# Autodesk Inventor assembly: 42146-19
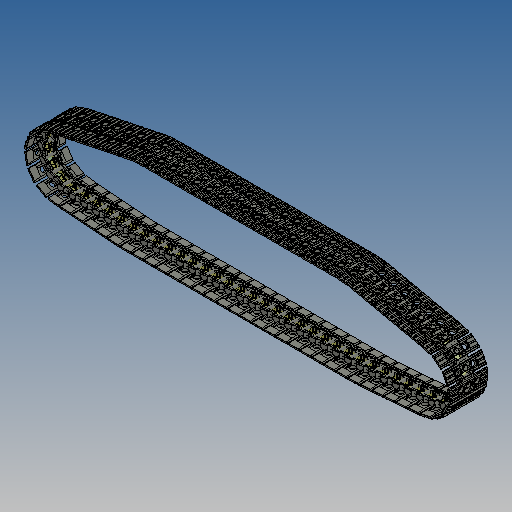
[picture p0: Inventor's stored thumbnail of the model, 512x512]
Saved by Autodesk Inventor 2025 (Build 290162010, 162A)
## iProperties
Created: 2024-11-19
Part Number: 42146-19
Material: Generisch
Document SubType Name: Assembly
Designer: hp.muther
Author: hp.muther
## Documents named in this file (3)
- D:\Inventor\Projekte\Muther\LEGO Technic\LEGO Technik - Raupenkran LR 13000 (42146)\42146-19.iam
- D:\Inventor\Projekte\Muther\LEGO Technic\LEGO Technik - Raupenkran LR 13000 (42146)\42146-19.ipt
- D:\Inventor\Projekte\Muther\LEGO Technic\LEGO Pieces\Räder, Raupe\57518-DkBluishGray.ipt
## Components (76 placed, 2 different names)
1. 42146-19:1 — Passend:1, Passend:2, Passend:3, Passend:4, Passend:5, Passend:6, Passend:7, Tangential:1, Tangential:2, Tangential:3, Tangential:4, Tangential:5, Tangential:6, Passend:8, Passend:9, Passend:10, Passend:11, Passend:12, Passend:13, Passend:14, Passend:15, Passend:16, Passend:17, Passend:18, Passend:19, Passend:20, Passend:21, Passend:22, Passend:23, Passend:24, Passend:25, Passend:26, Passend:27, Passend:28, Passend:29, Passend:30, Passend:31, Passend:32, Passend:33, Passend:34, Passend:35, Passend:36, Passend:37, Passend:38, Passend:39, Passend:40, Tangential:7, Tangential:8, Tangential:9, Tangential:10, Tangential:11, Tangential:12, Passend:41, Passend:42, Passend:43, Passend:44, Passend:45, Passend:46, Passend:47, Passend:48, Passend:49, Passend:50, Passend:51, Passend:52, Passend:53, Passend:54, Passend:55, Passend:56, Passend:57, Passend:58, Passend:59, Passend:60, Passend:61, Passend:62, Passend:63, Passend:64, Passend:65
2. 57518-DkBluishGray:1 — Passend:1, Passend:2, Passend:3, Einfügen:1
3. 57518-DkBluishGray:2 — Einfügen:1, Einfügen:3, Passend:4
4. 57518-DkBluishGray:3 — Einfügen:3, Passend:5
5. 57518-DkBluishGray:4 — Einfügen:7, Passend:6
6. 57518-DkBluishGray:5 — Einfügen:7, Passend:7
7. 57518-DkBluishGray:6 — Passend:10
8. 57518-DkBluishGray:7 — Tangential:1
9. 57518-DkBluishGray:8 — Einfügen:15, Tangential:2
10. 57518-DkBluishGray:9 — Einfügen:15, Tangential:3
11. 57518-DkBluishGray:10 — Tangential:4
12. 57518-DkBluishGray:11 — Tangential:5
13. 57518-DkBluishGray:12 — Tangential:6
14. 57518-DkBluishGray:13 — Passend:8
15. 57518-DkBluishGray:14 — Passend:9
16. 57518-DkBluishGray:15 — Passend:11
17. 57518-DkBluishGray:16 — Passend:12, Einfügen:31
18. 57518-DkBluishGray:17 — Einfügen:31, Passend:13
19. 57518-DkBluishGray:18 — Passend:14
20. 57518-DkBluishGray:19 — Passend:15
21. 57518-DkBluishGray:20 — Passend:16
22. 57518-DkBluishGray:21 — Passend:17
23. 57518-DkBluishGray:22 — Passend:18
24. 57518-DkBluishGray:23 — Passend:19
25. 57518-DkBluishGray:24 — Passend:20
26. 57518-DkBluishGray:25 — Passend:21
27. 57518-DkBluishGray:26 — Passend:22
28. 57518-DkBluishGray:27 — Passend:23
29. 57518-DkBluishGray:28 — Passend:24
30. 57518-DkBluishGray:29 — Passend:25
31. 57518-DkBluishGray:30 — Passend:26
32. 57518-DkBluishGray:31 — Passend:27
33. 57518-DkBluishGray:32 — Passend:28, Einfügen:63
34. 57518-DkBluishGray:33 — Einfügen:63, Passend:29
35. 57518-DkBluishGray:34 — Passend:30
36. 57518-DkBluishGray:35 — Passend:31
37. 57518-DkBluishGray:36 — Passend:32
38. 57518-DkBluishGray:37 — Passend:33
39. 57518-DkBluishGray:38 — Passend:34
40. 57518-DkBluishGray:39 — Passend:35
41. 57518-DkBluishGray:40 — Passend:36
42. 57518-DkBluishGray:41 — Passend:37
43. 57518-DkBluishGray:42 — Passend:38
44. 57518-DkBluishGray:43 — Passend:39
45. 57518-DkBluishGray:44 — Passend:40
46. 57518-DkBluishGray:45 — Tangential:7
47. 57518-DkBluishGray:46 — Tangential:8
48. 57518-DkBluishGray:47 — Tangential:9
49. 57518-DkBluishGray:48 — Tangential:10
50. 57518-DkBluishGray:49 — Tangential:11
51. 57518-DkBluishGray:50 — Tangential:12
52. 57518-DkBluishGray:51 — Passend:41
53. 57518-DkBluishGray:52 — Passend:42
54. 57518-DkBluishGray:53 — Passend:43
55. 57518-DkBluishGray:54 — Passend:44
56. 57518-DkBluishGray:55 — Passend:45
57. 57518-DkBluishGray:56 — Passend:46
58. 57518-DkBluishGray:57 — Passend:47
59. 57518-DkBluishGray:58 — Passend:48
60. 57518-DkBluishGray:59 — Passend:49
61. 57518-DkBluishGray:60 — Passend:50
62. 57518-DkBluishGray:61 — Passend:51
63. 57518-DkBluishGray:62 — Passend:52
64. 57518-DkBluishGray:63 — Passend:53
65. 57518-DkBluishGray:64 — Passend:54, Einfügen:75
66. 57518-DkBluishGray:65 — Einfügen:75, Passend:55
67. 57518-DkBluishGray:66 — Passend:56
68. 57518-DkBluishGray:67 — Passend:57
69. 57518-DkBluishGray:68 — Passend:58
70. 57518-DkBluishGray:69 — Passend:59
71. 57518-DkBluishGray:70 — Passend:61
72. 57518-DkBluishGray:71 — Passend:60
73. 57518-DkBluishGray:72 — Passend:62
74. 57518-DkBluishGray:73 — Passend:63
75. 57518-DkBluishGray:74 — Passend:64
76. 57518-DkBluishGray:75 — Passend:65
## Relationships (151: Insert 74, Mate 65, Tangent 12)
- Passend:1 [Mate] (-19.2 mm): 42146-19:1 ↔ 57518-DkBluishGray:1
- Passend:2 [Mate]: 42146-19:1 ↔ 57518-DkBluishGray:1
- Passend:3 [Mate]: 42146-19:1 ↔ 57518-DkBluishGray:1
- Einfügen:1 [Insert]: 57518-DkBluishGray:1 ↔ 57518-DkBluishGray:2
- [Insert]: 57518-DkBluishGray:3 ↔ 57518-DkBluishGray:4
- Einfügen:3 [Insert]: 57518-DkBluishGray:2 ↔ 57518-DkBluishGray:3
- [Insert]: 57518-DkBluishGray:5 ↔ 57518-DkBluishGray:6
- [Insert]: 57518-DkBluishGray:7 ↔ 57518-DkBluishGray:8
- [Insert]: 57518-DkBluishGray:6 ↔ 57518-DkBluishGray:7
- Einfügen:7 [Insert]: 57518-DkBluishGray:4 ↔ 57518-DkBluishGray:5
- [Insert]: 57518-DkBluishGray:9 ↔ 57518-DkBluishGray:10
- [Insert]: 57518-DkBluishGray:11 ↔ 57518-DkBluishGray:12
- [Insert]: 57518-DkBluishGray:10 ↔ 57518-DkBluishGray:11
- [Insert]: 57518-DkBluishGray:13 ↔ 57518-DkBluishGray:14
- [Insert]: 57518-DkBluishGray:15 ↔ 57518-DkBluishGray:16
- [Insert]: 57518-DkBluishGray:14 ↔ 57518-DkBluishGray:15
- [Insert]: 57518-DkBluishGray:12 ↔ 57518-DkBluishGray:13
- Einfügen:15 [Insert]: 57518-DkBluishGray:8 ↔ 57518-DkBluishGray:9
- Passend:4 [Mate]: 42146-19:1 ↔ 57518-DkBluishGray:2
- Passend:5 [Mate]: 42146-19:1 ↔ 57518-DkBluishGray:3
- Passend:6 [Mate]: 42146-19:1 ↔ 57518-DkBluishGray:4
- Passend:7 [Mate]: 42146-19:1 ↔ 57518-DkBluishGray:5
- Tangential:1 (-1.6 mm): 42146-19:1 ↔ 57518-DkBluishGray:7
- Tangential:2 (-1.6 mm): 42146-19:1 ↔ 57518-DkBluishGray:8
- Tangential:3 (-1.6 mm): 42146-19:1 ↔ 57518-DkBluishGray:9
- Tangential:4 (-1.6 mm): 42146-19:1 ↔ 57518-DkBluishGray:10
- Tangential:5 (-1.6 mm): 42146-19:1 ↔ 57518-DkBluishGray:11
- Tangential:6 (-1.6 mm): 42146-19:1 ↔ 57518-DkBluishGray:12
- Passend:8 [Mate]: 42146-19:1 ↔ 57518-DkBluishGray:13
- Passend:9 [Mate]: 42146-19:1 ↔ 57518-DkBluishGray:14
- Passend:10 [Mate]: 42146-19:1 ↔ 57518-DkBluishGray:6
- Passend:11 [Mate]: 42146-19:1 ↔ 57518-DkBluishGray:15
- Passend:12 [Mate]: 42146-19:1 ↔ 57518-DkBluishGray:16
- [Insert]: 57518-DkBluishGray:17 ↔ 57518-DkBluishGray:18
- [Insert]: 57518-DkBluishGray:19 ↔ 57518-DkBluishGray:20
- [Insert]: 57518-DkBluishGray:18 ↔ 57518-DkBluishGray:19
- [Insert]: 57518-DkBluishGray:21 ↔ 57518-DkBluishGray:22
- [Insert]: 57518-DkBluishGray:23 ↔ 57518-DkBluishGray:24
- [Insert]: 57518-DkBluishGray:22 ↔ 57518-DkBluishGray:23
- [Insert]: 57518-DkBluishGray:20 ↔ 57518-DkBluishGray:21
- [Insert]: 57518-DkBluishGray:25 ↔ 57518-DkBluishGray:26
- [Insert]: 57518-DkBluishGray:27 ↔ 57518-DkBluishGray:28
- [Insert]: 57518-DkBluishGray:26 ↔ 57518-DkBluishGray:27
- [Insert]: 57518-DkBluishGray:29 ↔ 57518-DkBluishGray:30
- [Insert]: 57518-DkBluishGray:31 ↔ 57518-DkBluishGray:32
- [Insert]: 57518-DkBluishGray:30 ↔ 57518-DkBluishGray:31
- [Insert]: 57518-DkBluishGray:28 ↔ 57518-DkBluishGray:29
- [Insert]: 57518-DkBluishGray:24 ↔ 57518-DkBluishGray:25
- Einfügen:31 [Insert]: 57518-DkBluishGray:16 ↔ 57518-DkBluishGray:17
- Passend:13 [Mate]: 42146-19:1 ↔ 57518-DkBluishGray:17
- Passend:14 [Mate]: 42146-19:1 ↔ 57518-DkBluishGray:18
- Passend:15 [Mate]: 42146-19:1 ↔ 57518-DkBluishGray:19
- Passend:16 [Mate]: 42146-19:1 ↔ 57518-DkBluishGray:20
- Passend:17 [Mate]: 42146-19:1 ↔ 57518-DkBluishGray:21
- Passend:18 [Mate]: 42146-19:1 ↔ 57518-DkBluishGray:22
- Passend:19 [Mate]: 42146-19:1 ↔ 57518-DkBluishGray:23
- Passend:20 [Mate]: 42146-19:1 ↔ 57518-DkBluishGray:24
- Passend:21 [Mate]: 42146-19:1 ↔ 57518-DkBluishGray:25
- Passend:22 [Mate]: 42146-19:1 ↔ 57518-DkBluishGray:26
- Passend:23 [Mate]: 42146-19:1 ↔ 57518-DkBluishGray:27
- Passend:24 [Mate]: 42146-19:1 ↔ 57518-DkBluishGray:28
- Passend:25 [Mate]: 42146-19:1 ↔ 57518-DkBluishGray:29
- Passend:26 [Mate]: 42146-19:1 ↔ 57518-DkBluishGray:30
- Passend:27 [Mate]: 42146-19:1 ↔ 57518-DkBluishGray:31
- Passend:28 [Mate]: 42146-19:1 ↔ 57518-DkBluishGray:32
- [Insert]: 57518-DkBluishGray:33 ↔ 57518-DkBluishGray:34
- [Insert]: 57518-DkBluishGray:35 ↔ 57518-DkBluishGray:36
- [Insert]: 57518-DkBluishGray:34 ↔ 57518-DkBluishGray:35
- [Insert]: 57518-DkBluishGray:37 ↔ 57518-DkBluishGray:38
- [Insert]: 57518-DkBluishGray:39 ↔ 57518-DkBluishGray:40
- [Insert]: 57518-DkBluishGray:38 ↔ 57518-DkBluishGray:39
- [Insert]: 57518-DkBluishGray:36 ↔ 57518-DkBluishGray:37
- [Insert]: 57518-DkBluishGray:41 ↔ 57518-DkBluishGray:42
- [Insert]: 57518-DkBluishGray:43 ↔ 57518-DkBluishGray:44
- [Insert]: 57518-DkBluishGray:42 ↔ 57518-DkBluishGray:43
- [Insert]: 57518-DkBluishGray:45 ↔ 57518-DkBluishGray:46
- [Insert]: 57518-DkBluishGray:47 ↔ 57518-DkBluishGray:48
- [Insert]: 57518-DkBluishGray:46 ↔ 57518-DkBluishGray:47
- [Insert]: 57518-DkBluishGray:44 ↔ 57518-DkBluishGray:45
- [Insert]: 57518-DkBluishGray:40 ↔ 57518-DkBluishGray:41
- [Insert]: 57518-DkBluishGray:49 ↔ 57518-DkBluishGray:50
- [Insert]: 57518-DkBluishGray:51 ↔ 57518-DkBluishGray:52
- [Insert]: 57518-DkBluishGray:50 ↔ 57518-DkBluishGray:51
- [Insert]: 57518-DkBluishGray:53 ↔ 57518-DkBluishGray:54
- [Insert]: 57518-DkBluishGray:55 ↔ 57518-DkBluishGray:56
- [Insert]: 57518-DkBluishGray:54 ↔ 57518-DkBluishGray:55
- [Insert]: 57518-DkBluishGray:52 ↔ 57518-DkBluishGray:53
- [Insert]: 57518-DkBluishGray:57 ↔ 57518-DkBluishGray:58
- [Insert]: 57518-DkBluishGray:59 ↔ 57518-DkBluishGray:60
- [Insert]: 57518-DkBluishGray:58 ↔ 57518-DkBluishGray:59
- [Insert]: 57518-DkBluishGray:61 ↔ 57518-DkBluishGray:62
- [Insert]: 57518-DkBluishGray:63 ↔ 57518-DkBluishGray:64
- [Insert]: 57518-DkBluishGray:62 ↔ 57518-DkBluishGray:63
- [Insert]: 57518-DkBluishGray:60 ↔ 57518-DkBluishGray:61
- [Insert]: 57518-DkBluishGray:56 ↔ 57518-DkBluishGray:57
- [Insert]: 57518-DkBluishGray:48 ↔ 57518-DkBluishGray:49
- Einfügen:63 [Insert]: 57518-DkBluishGray:32 ↔ 57518-DkBluishGray:33
- Passend:29 [Mate]: 42146-19:1 ↔ 57518-DkBluishGray:33
- Passend:30 [Mate]: 42146-19:1 ↔ 57518-DkBluishGray:34
- Passend:31 [Mate]: 42146-19:1 ↔ 57518-DkBluishGray:35
- Passend:32 [Mate]: 42146-19:1 ↔ 57518-DkBluishGray:36
- Passend:33 [Mate]: 42146-19:1 ↔ 57518-DkBluishGray:37
- Passend:34 [Mate]: 42146-19:1 ↔ 57518-DkBluishGray:38
- Passend:35 [Mate]: 42146-19:1 ↔ 57518-DkBluishGray:39
- Passend:36 [Mate]: 42146-19:1 ↔ 57518-DkBluishGray:40
- Passend:37 [Mate]: 42146-19:1 ↔ 57518-DkBluishGray:41
- Passend:38 [Mate]: 42146-19:1 ↔ 57518-DkBluishGray:42
- Passend:39 [Mate]: 42146-19:1 ↔ 57518-DkBluishGray:43
- Passend:40 [Mate]: 42146-19:1 ↔ 57518-DkBluishGray:44
- Tangential:7 (-1.6 mm): 42146-19:1 ↔ 57518-DkBluishGray:45
- Tangential:8 (-1.6 mm): 42146-19:1 ↔ 57518-DkBluishGray:46
- Tangential:9 (-1.6 mm): 42146-19:1 ↔ 57518-DkBluishGray:47
- Tangential:10 (-1.6 mm): 42146-19:1 ↔ 57518-DkBluishGray:48
- Tangential:11 (-1.6 mm): 42146-19:1 ↔ 57518-DkBluishGray:49
- Tangential:12 (-1.6 mm): 42146-19:1 ↔ 57518-DkBluishGray:50
- Passend:41 [Mate]: 42146-19:1 ↔ 57518-DkBluishGray:51
- Passend:42 [Mate]: 42146-19:1 ↔ 57518-DkBluishGray:52
- Passend:43 [Mate]: 42146-19:1 ↔ 57518-DkBluishGray:53
- Passend:44 [Mate]: 42146-19:1 ↔ 57518-DkBluishGray:54
- Passend:45 [Mate]: 42146-19:1 ↔ 57518-DkBluishGray:55
- Passend:46 [Mate]: 42146-19:1 ↔ 57518-DkBluishGray:56
- Passend:47 [Mate]: 42146-19:1 ↔ 57518-DkBluishGray:57
- Passend:48 [Mate]: 42146-19:1 ↔ 57518-DkBluishGray:58
- Passend:49 [Mate]: 42146-19:1 ↔ 57518-DkBluishGray:59
- Passend:50 [Mate]: 42146-19:1 ↔ 57518-DkBluishGray:60
- Passend:51 [Mate]: 42146-19:1 ↔ 57518-DkBluishGray:61
- Passend:52 [Mate]: 42146-19:1 ↔ 57518-DkBluishGray:62
- Passend:53 [Mate]: 42146-19:1 ↔ 57518-DkBluishGray:63
- Passend:54 [Mate]: 42146-19:1 ↔ 57518-DkBluishGray:64
- [Insert]: 57518-DkBluishGray:65 ↔ 57518-DkBluishGray:66
- [Insert]: 57518-DkBluishGray:67 ↔ 57518-DkBluishGray:68
- [Insert]: 57518-DkBluishGray:66 ↔ 57518-DkBluishGray:67
- [Insert]: 57518-DkBluishGray:69 ↔ 57518-DkBluishGray:70
- [Insert]: 57518-DkBluishGray:71 ↔ 57518-DkBluishGray:72
- [Insert]: 57518-DkBluishGray:70 ↔ 57518-DkBluishGray:71
- [Insert]: 57518-DkBluishGray:73 ↔ 57518-DkBluishGray:74
- [Insert]: 57518-DkBluishGray:74 ↔ 57518-DkBluishGray:75
- [Insert]: 57518-DkBluishGray:72 ↔ 57518-DkBluishGray:73
- [Insert]: 57518-DkBluishGray:68 ↔ 57518-DkBluishGray:69
- Einfügen:75 [Insert]: 57518-DkBluishGray:64 ↔ 57518-DkBluishGray:65
- Passend:55 [Mate]: 42146-19:1 ↔ 57518-DkBluishGray:65
- Passend:56 [Mate]: 42146-19:1 ↔ 57518-DkBluishGray:66
- Passend:57 [Mate]: 42146-19:1 ↔ 57518-DkBluishGray:67
- Passend:58 [Mate]: 42146-19:1 ↔ 57518-DkBluishGray:68
- Passend:59 [Mate]: 42146-19:1 ↔ 57518-DkBluishGray:69
- Passend:60 [Mate]: 42146-19:1 ↔ 57518-DkBluishGray:71
- Passend:61 [Mate]: 42146-19:1 ↔ 57518-DkBluishGray:70
- Passend:62 [Mate]: 42146-19:1 ↔ 57518-DkBluishGray:72
- Passend:63 [Mate]: 42146-19:1 ↔ 57518-DkBluishGray:73
- Passend:64 [Mate]: 42146-19:1 ↔ 57518-DkBluishGray:74
- Passend:65 [Mate]: 42146-19:1 ↔ 57518-DkBluishGray:75
## Named parameters: d12_d11 = 0 mm, d14_d11 = 0 mm, d15_d12_d11 = 0 mm, d16_d13 = 0 mm, d18_d11 = 0 mm, d19_d12_d11 = 0 mm, d20_d13 = 0 mm, d21_d14_d11 = 0 mm, d22_d15_d12_d11 = 0 mm, d23_d16_d13 = 0 mm, d24_d17 = 0 mm, d41_d25 = 0 mm, d42_d11 = 0 mm, d43_d12_d11 = 0 mm, d44_d13 = 0 mm, d45_d14_d11 = 0 mm, d46_d15_d12_d11 = 0 mm, d47_d16_d13 = 0 mm, d48_d17 = 0 mm, d49_d18_d11 = 0 mm, d50_d19_d12_d11 = 0 mm, d51_d20_d13 = 0 mm, d52_d21_d14_d11 = 0 mm, d53_d22_d15_d12_d11 = 0 mm, d54_d23_d16_d13 = 0 mm, d55_d24_d17 = 0 mm, d73_d41_d25 = 0 mm, d74_d42_d11 = 0 mm, d75_d43_d12_d11 = 0 mm, d76_d44_d13 = 0 mm, d77_d45_d14_d11 = 0 mm, d78_d46_d15_d12_d11 = 0 mm, d79_d47_d16_d13 = 0 mm, d80_d48_d17 = 0 mm, d81_d49_d18_d11 = 0 mm, d82_d50_d19_d12_d11 = 0 mm, d83_d51_d20_d13 = 0 mm, d84_d52_d21_d14_d11 = 0 mm, d85_d53_d22_d15_d12_d11 = 0 mm, d86_d54_d23_d16_d13 = 0 mm, d87_d55_d24_d17 = 0 mm, d88_d56 = 0 mm, d89_d11 = 0 mm, d90_d12_d11 = 0 mm, d91_d13 = 0 mm, d92_d14_d11 = 0 mm, d93_d15_d12_d11 = 0 mm, d94_d16_d13 = 0 mm, d95_d17 = 0 mm, d96_d18_d11 = 0 mm, d97_d19_d12_d11 = 0 mm, d98_d20_d13 = 0 mm, d99_d21_d14_d11 = 0 mm, d100_d22_d15_d12_d11 = 0 mm, d101_d23_d16_d13 = 0 mm, d102_d24_d17 = 0 mm, d103_d25 = 0 mm, d137_d73_d41_d25 = 0 mm, d138_d77_d45_d14_d11 = 0 mm, d139_d78_d46_d15_d12_d11 = 0 mm, d140_d79_d47_d16_d13 = 0 mm, d141_d81_d49_d18_d11 = 0 mm, d142_d82_d50_d19_d12_d11 = 0 mm, d143_d83_d51_d20_d13 = 0 mm, d144_d84_d52_d21_d14_d11 = 0 mm, d146_d86_d54_d23_d16_d13 = 0 mm, d147_d87_d55_d24_d17 = 0 mm
